# Autodesk Inventor assembly: main assembly
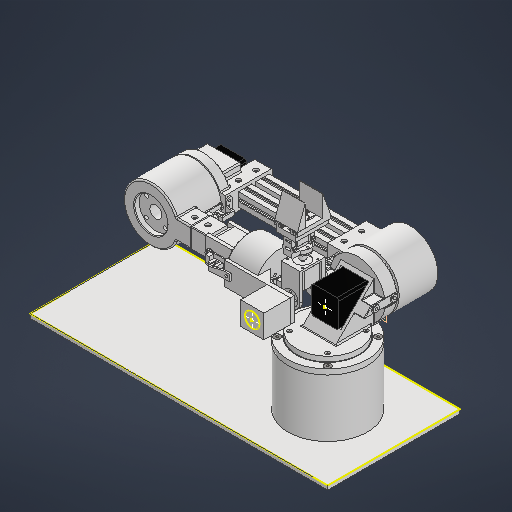
[picture p0: Inventor's stored thumbnail of the model, 512x512]
Saved by Autodesk Inventor 2026.1 (Build 301233020, 233B)
## iProperties
Created: 2025-07-04
Part Number: main assembly
Document SubType Name: Assembly
Designer: gavin
Author: gavin
## Documents named in this file (31)
- F:\temp data disk\Github\6-DOF-Robot-Arm\3D-model\robot armT 2(CAD file)\main assembly.iam
- F:\temp data disk\Github\6-DOF-Robot-Arm\3D-model\robot armT 2(CAD file)\stepper 42x48 - 27.ipt
- F:\temp data disk\Github\6-DOF-Robot-Arm\3D-model\robot armT 2(CAD file)\28stepper27.ipt
- F:\temp data disk\Github\6-DOF-Robot-Arm\3D-model\robot armT 2(CAD file)\CSN 02 4630 - 6009.ipt
- F:\temp data disk\Github\6-DOF-Robot-Arm\3D-model\robot armT 2(CAD file)\CNS 2862 B2116 - 6007 - 35 x 62 x 14.ipt
- F:\temp data disk\Github\6-DOF-Robot-Arm\3D-model\robot armT 2(CAD file)\base plate.ipt
- F:\temp data disk\Github\6-DOF-Robot-Arm\3D-model\robot armT 2(CAD file)\stepper 42x60 -50 .ipt
- F:\temp data disk\Github\6-DOF-Robot-Arm\3D-model\robot armT 2(CAD file)\j2 42 motor mount.ipt
- F:\temp data disk\Github\6-DOF-Robot-Arm\3D-model\robot armT 2(CAD file)\j1 assmble.iam
- F:\temp data disk\Github\6-DOF-Robot-Arm\3D-model\robot armT 2(CAD file)\optic endstop module.ipt
- F:\temp data disk\Github\6-DOF-Robot-Arm\3D-model\robot armT 2(CAD file)\j2j3 alumi ext.ipt
- F:\temp data disk\Github\6-DOF-Robot-Arm\3D-model\robot armT 2(CAD file)\j3 motor mount.ipt
- F:\temp data disk\Github\6-DOF-Robot-Arm\3D-model\robot armT 2(CAD file)\j3 moving part.ipt
- F:\temp data disk\Github\6-DOF-Robot-Arm\3D-model\robot armT 2(CAD file)\j3j4 alumi ext.ipt
- F:\temp data disk\Github\6-DOF-Robot-Arm\3D-model\robot armT 2(CAD file)\j2 endstop blocker.ipt
- F:\temp data disk\Github\6-DOF-Robot-Arm\3D-model\robot armT 2(CAD file)\j3 endstop blocker.ipt
- F:\temp data disk\Github\6-DOF-Robot-Arm\3D-model\robot armT 2(CAD file)\6mm axle hub.ipt
- F:\temp data disk\Github\6-DOF-Robot-Arm\3D-model\robot armT 2(CAD file)\j4 motor mount.ipt
- F:\temp data disk\Github\6-DOF-Robot-Arm\3D-model\robot armT 2(CAD file)\j4 motor mount cover.ipt
- F:\temp data disk\Github\6-DOF-Robot-Arm\3D-model\robot armT 2(CAD file)\j4 moving part.ipt
- F:\temp data disk\Github\6-DOF-Robot-Arm\3D-model\robot armT 2(CAD file)\nema 11x25.ipt
- F:\temp data disk\Github\6-DOF-Robot-Arm\3D-model\robot armT 2(CAD file)\5mm axle hub.ipt
- F:\temp data disk\Github\6-DOF-Robot-Arm\3D-model\robot armT 2(CAD file)\bearing 22-M6.ipt
- F:\temp data disk\Github\6-DOF-Robot-Arm\3D-model\robot armT 2(CAD file)\j6 motor mount v2.ipt
- F:\temp data disk\Github\6-DOF-Robot-Arm\3D-model\robot armT 2(CAD file)\j4 endstop blocker.ipt
- F:\temp data disk\Github\6-DOF-Robot-Arm\3D-model\robot armT 2(CAD file)\sg90 long claw.iam
- F:\temp data disk\Github\6-DOF-Robot-Arm\3D-model\robot armT 2(CAD file)\35x40 stepper.ipt
- F:\temp data disk\Github\6-DOF-Robot-Arm\3D-model\robot armT 2(CAD file)\j3 moving part option3.ipt
- F:\temp data disk\Github\6-DOF-Robot-Arm\3D-model\robot armT 2(CAD file)\z21 8x18.ipt
- F:\temp data disk\Github\6-DOF-Robot-Arm\3D-model\robot armT 2(CAD file)\18mm hub.ipt
- F:\temp data disk\Github\6-DOF-Robot-Arm\3D-model\robot armT 2(CAD file)\j2 moving part option2.ipt
## Components (38 placed, 30 different names)
1. base plate:1 — Flush:5
2. j1 assmble:1 [sub-assembly]
3. stepper 42x48 - 27:2 — Mate:45, Mate:46, Mate:47, Mate:110, Flush:18
4. CSN 02 4630 - 6009:1 — Mate:48, Mate:49, Mate:50, Mate:51, Mate:111, Flush:19
5. CSN 02 4630 - 6009:2 — Mate:16, Mate:29, Mate:114
6. CNS 2862 B2116 - 6007 - 35 x 62 x 14:1 — Mate:63, Mate:64, Mate:75, Flush:17
7. stepper 42x60 -50 :1 — Mate:16, Mate:27, Mate:28, Mate:113, Flush:20
8. j2 42 motor mount:1 — Mate:27, Mate:28, Mate:29, Mate:33, Mate:34, Mate:35
9. optic endstop module:1 — Mate:33, Mate:34, Mate:35, Flush:10
10. j2j3 alumi ext:1 — Mate:42, Mate:43, Mate:44, Flush:13
11. j2j3 alumi ext:2 — Mate:116
12. j3 motor mount:1 — Mate:42, Mate:43, Mate:44, Mate:45, Mate:46, Mate:47, Mate:48, Mate:49, Flush:11, Flush:12, Mate:59
13. j3 moving part:1 — Mate:50, Mate:51, Mate:52, Mate:53, Mate:54, Mate:55, Mate:56, Mate:57
14. j3j4 alumi ext:1 — Mate:52, Mate:53, Mate:54, Flush:13, Mate:68, Mate:69, Mate:70
15. optic endstop module:2 — Mate:55, Mate:56, Mate:57, Mate:58
16. j2 endstop blocker:1 — Flush:10
17. j3 endstop blocker:1 — Flush:11, Flush:12, Mate:58, Mate:59
18. 6mm axle hub:1 — Rotational:13, Mate:106
19. j4 motor mount:1 — Flush:14, Flush:15, Mate:60, Mate:61, Mate:62, Mate:63, Mate:65, Mate:68, Mate:69, Mate:70, Mate:71, Mate:72, Mate:73
20. j4 motor mount cover:1 — Flush:14, Flush:15, Mate:62, Mate:64, Mate:65
21. 28stepper27:1 — Mate:60, Mate:61, Rotational:13
22. optic endstop module:3 — Mate:71, Mate:72, Mate:73
23. j4 moving part:1 — Mate:74, Mate:75, Flush:17, Mate:76, Mate:86, Mate:87, Mate:104, Mate:105, Mate:106, Mate:107, Mate:108, Mate:109
24. nema 11x25:1 — Mate:88, Mate:89, Mate:102, Mate:103
25. optic endstop module:4 — Mate:74, Mate:76, Mate:107
26. 5mm axle hub:1 — Rigid:1, Rotational:12
27. bearing 22-M6:1 — Mate:86, Mate:87
28. j6 motor mount v2:1 — Mate:88, Mate:89, Rotational:12
29. j4 endstop blocker:1 — Mate:108, Mate:109
30. sg90 long claw:1 [sub-assembly] — Mate:99, Mate:100, Mate:101, Mate:103
31. 5mm axle hub:2 — Mate:99, Mate:100, Mate:101, Mate:102
32. 35x40 stepper:1 — Mate:104, Mate:105, Rigid:1
33. j3 moving part option3:1 — Mate:111, Flush:19, Mate:112
34. z21 8x18:1 — Rigid:2, Mate:110, Flush:18
35. 18mm hub:1 — Rigid:2, Mate:112
36. j2 moving part option2:1 — Mate:114, Mate:115, Mate:116
37. z21 8x18:2 — Mate:113, Flush:20
38. 18mm hub:2 — Mate:115
## Relationships (92: Mate 69, Flush 12, RevoluteJoint 8, WeldJoint 3)
- [Mate]: j1 assmble:1
- [Flush]: base plate:1 ↔ j1 assmble:1
- [Mate]: base plate:1 ↔ j1 assmble:1
- Flush:5: base plate:1
- Mate:16: CSN 02 4630 - 6009:2 ↔ stepper 42x60 -50 :1
- [Mate] (20 mm): j1 assmble:1 ↔ stepper 42x60 -50 :1
- [Mate]: j1 assmble:1 ↔ j2 42 motor mount:1
- [Mate]: base plate:1 ↔ j1 assmble:1
- [Mate]: j1 assmble:1 ↔ j2 42 motor mount:1
- [Mate]: j1 assmble:1 ↔ j2 42 motor mount:1
- Mate:27: stepper 42x60 -50 :1 ↔ j2 42 motor mount:1
- Mate:28: stepper 42x60 -50 :1 ↔ j2 42 motor mount:1
- Mate:29: CSN 02 4630 - 6009:2 ↔ j2 42 motor mount:1
- [RevoluteJoint]: base plate:1 ↔ j1 assmble:1
- [RevoluteJoint]: base plate:1 ↔ j1 assmble:1
- [RevoluteJoint]: base plate:1 ↔ j1 assmble:1
- [RevoluteJoint]: base plate:1 ↔ j1 assmble:1
- [RevoluteJoint]: base plate:1 ↔ j1 assmble:1
- [RevoluteJoint]: base plate:1 ↔ j1 assmble:1
- Mate:33: j2 42 motor mount:1 ↔ optic endstop module:1
- Mate:34: j2 42 motor mount:1 ↔ optic endstop module:1
- Mate:35: j2 42 motor mount:1 ↔ optic endstop module:1
- Mate:42: j2j3 alumi ext:1 ↔ j3 motor mount:1
- Mate:43 (0.075 mm): j2j3 alumi ext:1 ↔ j3 motor mount:1
- Mate:44 (0.075 mm): j2j3 alumi ext:1 ↔ j3 motor mount:1
- Mate:45: stepper 42x48 - 27:2 ↔ j3 motor mount:1
- Mate:46 (0.075 mm): stepper 42x48 - 27:2 ↔ j3 motor mount:1
- Mate:47: stepper 42x48 - 27:2 ↔ j3 motor mount:1
- Mate:48: CSN 02 4630 - 6009:1 ↔ j3 motor mount:1
- Mate:49: CSN 02 4630 - 6009:1 ↔ j3 motor mount:1
- Mate:50: CSN 02 4630 - 6009:1 ↔ j3 moving part:1
- Mate:51: CSN 02 4630 - 6009:1 ↔ j3 moving part:1
- Mate:52 (0.075 mm): j3 moving part:1 ↔ j3j4 alumi ext:1
- Mate:53: j3 moving part:1 ↔ j3j4 alumi ext:1
- Mate:54 (0.075 mm): j3 moving part:1 ↔ j3j4 alumi ext:1
- Mate:55: j3 moving part:1 ↔ optic endstop module:2
- Mate:56: j3 moving part:1 ↔ optic endstop module:2
- Mate:57: j3 moving part:1 ↔ optic endstop module:2
- Flush:10: optic endstop module:1 ↔ j2 endstop blocker:1
- Flush:11: j3 motor mount:1 ↔ j3 endstop blocker:1
- Flush:12: j3 motor mount:1 ↔ j3 endstop blocker:1
- Mate:58: optic endstop module:2 ↔ j3 endstop blocker:1
- Flush:13: j2j3 alumi ext:1 ↔ j3j4 alumi ext:1
- Flush:14: j4 motor mount:1 ↔ j4 motor mount cover:1
- Flush:15: j4 motor mount:1 ↔ j4 motor mount cover:1
- Mate:59: j3 motor mount:1 ↔ j3 endstop blocker:1
- Mate:60: j4 motor mount:1 ↔ 28stepper27:1
- Mate:61: j4 motor mount:1 ↔ 28stepper27:1
- Mate:62: j4 motor mount:1 ↔ j4 motor mount cover:1
- Mate:63: CNS 2862 B2116 - 6007 - 35 x 62 x 14:1 ↔ j4 motor mount:1
- Mate:64: CNS 2862 B2116 - 6007 - 35 x 62 x 14:1 ↔ j4 motor mount cover:1
- Mate:65: j4 motor mount:1 ↔ j4 motor mount cover:1
- Mate:68: j3j4 alumi ext:1 ↔ j4 motor mount:1
- Mate:69 (0.075 mm): j3j4 alumi ext:1 ↔ j4 motor mount:1
- Mate:70 (0.075 mm): j3j4 alumi ext:1 ↔ j4 motor mount:1
- Mate:71: j4 motor mount:1 ↔ optic endstop module:3
- Mate:72: j4 motor mount:1 ↔ optic endstop module:3
- Mate:73: j4 motor mount:1 ↔ optic endstop module:3
- Mate:74: j4 moving part:1 ↔ optic endstop module:4
- Mate:75: CNS 2862 B2116 - 6007 - 35 x 62 x 14:1 ↔ j4 moving part:1
- Flush:17: CNS 2862 B2116 - 6007 - 35 x 62 x 14:1 ↔ j4 moving part:1
- Mate:76: j4 moving part:1 ↔ optic endstop module:4
- Mate:86: j4 moving part:1 ↔ bearing 22-M6:1
- Mate:87: j4 moving part:1 ↔ bearing 22-M6:1
- Mate:88: nema 11x25:1 ↔ j6 motor mount v2:1
- Mate:89: nema 11x25:1 ↔ j6 motor mount v2:1
- Mate:99: sg90 long claw:1 ↔ 5mm axle hub:2
- Mate:100: sg90 long claw:1 ↔ 5mm axle hub:2
- Mate:101: sg90 long claw:1 ↔ 5mm axle hub:2
- Mate:102: nema 11x25:1 ↔ 5mm axle hub:2
- Mate:103: nema 11x25:1 ↔ sg90 long claw:1
- Mate:104: j4 moving part:1 ↔ 35x40 stepper:1
- Mate:105: j4 moving part:1 ↔ 35x40 stepper:1
- Rigid:1 [WeldJoint]: 5mm axle hub:1 ↔ 35x40 stepper:1
- Rotational:12 [RevoluteJoint]: 5mm axle hub:1 ↔ j6 motor mount v2:1
- Rotational:13 [RevoluteJoint]: 6mm axle hub:1 ↔ 28stepper27:1
- Mate:106: 6mm axle hub:1 ↔ j4 moving part:1
- Mate:107: j4 moving part:1 ↔ optic endstop module:4
- Mate:108: j4 moving part:1 ↔ j4 endstop blocker:1
- Mate:109: j4 moving part:1 ↔ j4 endstop blocker:1
- Rigid:2 [WeldJoint] (-3.71 mm): z21 8x18:1 ↔ 18mm hub:1
- Mate:110: stepper 42x48 - 27:2 ↔ z21 8x18:1
- Flush:18: stepper 42x48 - 27:2 ↔ z21 8x18:1
- Mate:111: CSN 02 4630 - 6009:1 ↔ j3 moving part option3:1
- Flush:19: CSN 02 4630 - 6009:1 ↔ j3 moving part option3:1
- Mate:112: j3 moving part option3:1 ↔ 18mm hub:1
- [WeldJoint] (-3.71 mm): z21 8x18:2 ↔ 18mm hub:2
- Mate:113: stepper 42x60 -50 :1 ↔ z21 8x18:2
- Flush:20: stepper 42x60 -50 :1 ↔ z21 8x18:2
- Mate:114: CSN 02 4630 - 6009:2 ↔ j2 moving part option2:1
- Mate:115: j2 moving part option2:1 ↔ 18mm hub:2
- Mate:116 (0.075 mm): j2j3 alumi ext:2 ↔ j2 moving part option2:1
## Named parameters: d225_d219 = -3.71 mm
